# Autodesk Inventor assembly: リンク_6_1
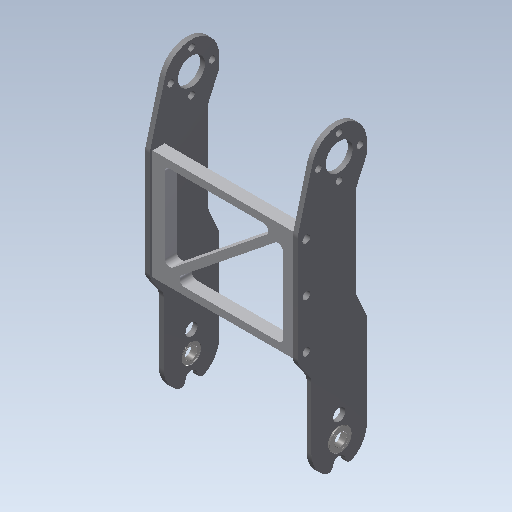
[picture p0: Inventor's stored thumbnail of the model, 512x512]
Saved by Autodesk Inventor 2020 (Build 240168000, 168)
## iProperties
Created: 2016-08-23
Part Number: リンク_6_1
Material: 一般
Document SubType Name: Assembly
Designer: hiro
Mass: 33.5175 g
Surface Area: 182.778 cm^2
Volume: 15.549 cm^3
Density: 2.15561 g/cm^3
Author: hiro
## Documents named in this file (4)
- C:\Inventor\OpenPlatform_ver3_0\下半身_160823\リンク\リンク_6_2.iam
- C:\Inventor\OpenPlatform_ver3_0\既製品\NSK_RB_MF85ZZ\MF85ZZ.iam
- C:\Inventor\OpenPlatform_ver3_0\下半身\リンク\ふくらはぎ\リンク_ふくらはぎ_サブフレーム_1_1(予備案).ipt
- C:\Inventor\OpenPlatform_ver3_0\下半身_160823\リンク\リンク_メインフレーム_6_4.ipt
## Components (5 placed, 3 different names)
1. MF85ZZ:1 [sub-assembly] — 挿入:6
2. MF85ZZ:2 [sub-assembly] — 挿入:5
3. リンク_ふくらはぎ_サブフレーム_1_1(予備案):1 — 挿入:1, 挿入:2, 挿入:3, 挿入:4
4. リンク_メインフレーム_6_4:1 — 挿入:1, 挿入:2, 挿入:6
5. リンク_メインフレーム_6_4:2 — 挿入:3, 挿入:4, 挿入:5
## Relationships (6: Insert 6)
- 挿入:1 [Insert]: リンク_ふくらはぎ_サブフレーム_1_1(予備案):1 ↔ リンク_メインフレーム_6_4:1
- 挿入:2 [Insert]: リンク_ふくらはぎ_サブフレーム_1_1(予備案):1 ↔ リンク_メインフレーム_6_4:1
- 挿入:3 [Insert]: リンク_ふくらはぎ_サブフレーム_1_1(予備案):1 ↔ リンク_メインフレーム_6_4:2
- 挿入:4 [Insert]: リンク_ふくらはぎ_サブフレーム_1_1(予備案):1 ↔ リンク_メインフレーム_6_4:2
- 挿入:5 [Insert]: MF85ZZ:2 ↔ リンク_メインフレーム_6_4:2
- 挿入:6 [Insert]: MF85ZZ:1 ↔ リンク_メインフレーム_6_4:1
